# Autodesk Inventor assembly: pir-hc-sr-501-sensor
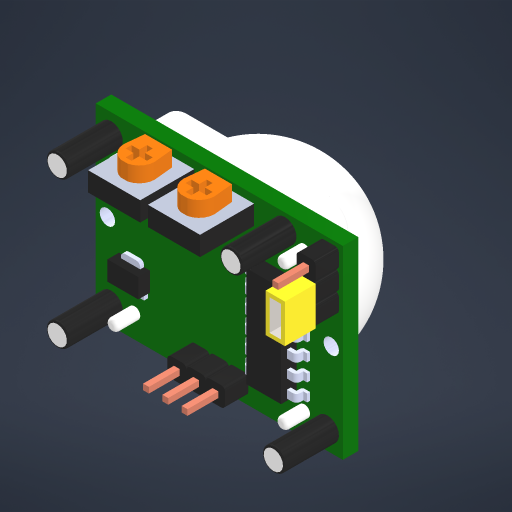
[picture p0: Inventor's stored thumbnail of the model, 512x512]
Saved by Autodesk Inventor 2023 (Build 270158000, 158)
## iProperties
Created: 2022-11-20
Part Number: pir-hc-sr-501-sensor
Document SubType Name: Assembly
Designer: Manuel
Author: Manuel
## Documents named in this file (3)
- C:\workspace\Studium\WST\opcua_netzwerk\Sensorknoten\3D Modell\pir-hc-sr-501-sensor\pir-hc-sr-501-sensor.iam
- C:\workspace\Studium\WST\opcua_netzwerk\Sensorknoten\3D Modell\pir-hc-sr-501-sensor\lens.ipt
- C:\workspace\Studium\WST\opcua_netzwerk\Sensorknoten\3D Modell\pir-hc-sr-501-sensor\sensor board.ipt
## Components (2 placed, 2 different names)
1. lens:1 — Passend:1, Passend:2, Passend:3
2. sensor board:1 — Passend:1, Passend:2, Passend:3
## Relationships (3: Mate 3)
- Passend:1 [Mate]: lens:1 ↔ sensor board:1
- Passend:2 [Mate]: lens:1 ↔ sensor board:1
- Passend:3 [Mate]: lens:1 ↔ sensor board:1
